# Autodesk Inventor assembly: GuiaLinealHGH20CA2T1050Z0H_FILE_1
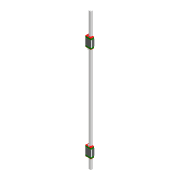
[picture p0: Inventor's stored thumbnail of the model, 180x180]
Saved by Autodesk Inventor 2021 (Build 250183000, 183)
## iProperties
Company: CADClick - www.CADClick.com
Created: 2021-08-22
Part Number: GuiaLinealHGH20CA2T1050Z0H_FILE_1
Description: STEP AP214
Document SubType Name: Assembly
Designer: Santiago Suárez
Authority: unknown authorization
Title: cctmp_0739CAEE-9F09-4F6F-BD52-DCFDED70B6C8_2021_08_22_06_56_33_0332..stp
Author: HIWIN GmbH
Revision Number: NONE
Preprocessor: Spatial InterOp 3D
## Documents named in this file (4)
- C:\Users\Santiago Suárez\Documents\GitHub\Dis.-Mecatronico-E6\inventor proyecto\Guias\GuiaLinealHGH20CA2T1050Z0H_FILE_1.iam
- C:\Users\Santiago Suárez\Documents\GitHub\Dis.-Mecatronico-E6\inventor proyecto\Guias\GuiaLinealHGH20CA2T1050Z0H_FILE_2.ipt
- C:\Users\Santiago Suárez\Documents\GitHub\Dis.-Mecatronico-E6\inventor proyecto\Guias\GuiaLinealHGH20CA2T1050Z0H_FILE_1.ipt
- C:\Users\Santiago Suárez\Documents\GitHub\Dis.-Mecatronico-E6\inventor proyecto\Guias\GuiaLinealHGH20CA2T1050Z0H_FILE.ipt
## Components (3 placed, 3 different names)
1. GuiaLinealHGH20CA2T1050Z0H_FILE_2 — Slider:2
2. GuiaLinealHGH20CA2T1050Z0H_FILE_1 — Slider:1
3. GuiaLinealHGH20CA2T1050Z0H_FILE — Slider:1, Slider:2
## Relationships (2: TranslationJoint 2)
- Slider:1 [TranslationJoint]: GuiaLinealHGH20CA2T1050Z0H_FILE_1 ↔ GuiaLinealHGH20CA2T1050Z0H_FILE
- Slider:2 [TranslationJoint]: GuiaLinealHGH20CA2T1050Z0H_FILE_2 ↔ GuiaLinealHGH20CA2T1050Z0H_FILE
